# Autodesk Inventor assembly: electronics-switch_perfboard
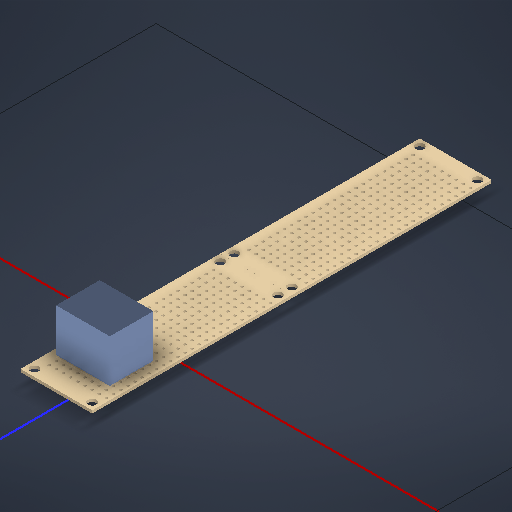
[picture p0: Inventor's stored thumbnail of the model, 512x512]
Saved by Autodesk Inventor 2025.2 (Build 292293000, 293)
## iProperties
Created: 2025-11-15
Part Number: electronics-switch_perfboard
Document SubType Name: Assembly
Designer: sam
Author: sam
## Documents named in this file (3)
- G:\projects\primary\auto-water-distribution-system\model\asm\module-switch\electronics-switch_perfboard.iam
- G:\projects\primary\auto-water-distribution-system\model\asm\general\perfboard-71x25.5x1_halfed.ipt
- G:\projects\primary\auto-water-distribution-system\model\asm\module-switch\electronic-components\relay_sdr-03vdc-sl-c.ipt
## Components (3 placed, 2 different names)
1. perfboard-71x25.5x1_halfed:1 — Mate:1, Flush:1, Flush:2, Mate:2, Mate:3, Mate:4
2. perfboard-71x25.5x1_halfed:2 — Mate:1, Flush:1, Flush:2
3. relay_sdr-03vdc-sl-c:1 — Mate:2, Mate:3, Mate:4
## Relationships (6: Mate 4, Flush 2)
- Mate:1: perfboard-71x25.5x1_halfed:1 ↔ perfboard-71x25.5x1_halfed:2
- Flush:1: perfboard-71x25.5x1_halfed:1 ↔ perfboard-71x25.5x1_halfed:2
- Flush:2: perfboard-71x25.5x1_halfed:1 ↔ perfboard-71x25.5x1_halfed:2
- Mate:2: perfboard-71x25.5x1_halfed:1 ↔ relay_sdr-03vdc-sl-c:1
- Mate:3: perfboard-71x25.5x1_halfed:1 ↔ relay_sdr-03vdc-sl-c:1
- Mate:4 (1 mm): perfboard-71x25.5x1_halfed:1 ↔ relay_sdr-03vdc-sl-c:1
